# Autodesk Inventor assembly: PumpMount_wSwitch_v03
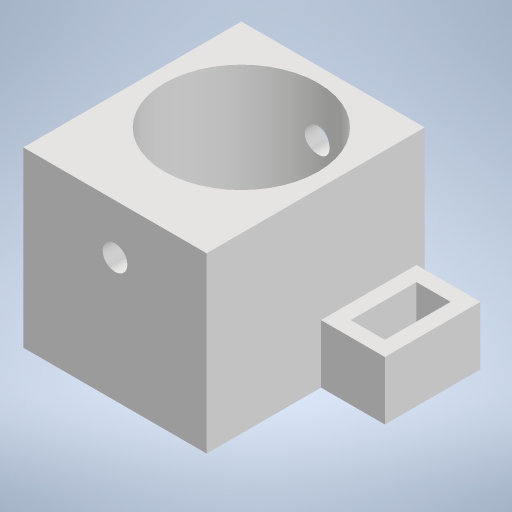
[picture p0: Inventor's stored thumbnail of the model, 512x512]
Saved by Autodesk Inventor 2023.5 (Build 275446000, 446)
## iProperties
Created: 2024-08-19
Part Number: PumpMount_wSwitch_v03
Document SubType Name: Assembly
Designer: Akramilab
Author: Akramilab
## Documents named in this file (3)
- C:\Projects\Inventor\Touchscreen arena\Pump mount\PumpMount_wSwitch_v03.iam
- C:\Projects\Inventor\Touchscreen arena\Pump mount\switch test v02b.ipt
- C:\Projects\Inventor\Touchscreen arena\Pump mount\pump mount v04.ipt
## Components (2 placed, 2 different names)
1. switch test v02b:1 — Flush:1, Mate:1, Flush:2, Mate:2, Flush:3
2. pump mount v04:1 — Flush:1, Mate:1, Flush:2, Mate:2, Flush:3
## Relationships (5: Flush 3, Mate 2)
- Flush:1: switch test v02b:1 ↔ pump mount v04:1
- Mate:1: switch test v02b:1 ↔ pump mount v04:1
- Flush:2: switch test v02b:1 ↔ pump mount v04:1
- Mate:2: switch test v02b:1 ↔ pump mount v04:1
- Flush:3: switch test v02b:1 ↔ pump mount v04:1
